# Autodesk Inventor assembly: Leg_joint_roll_yaw
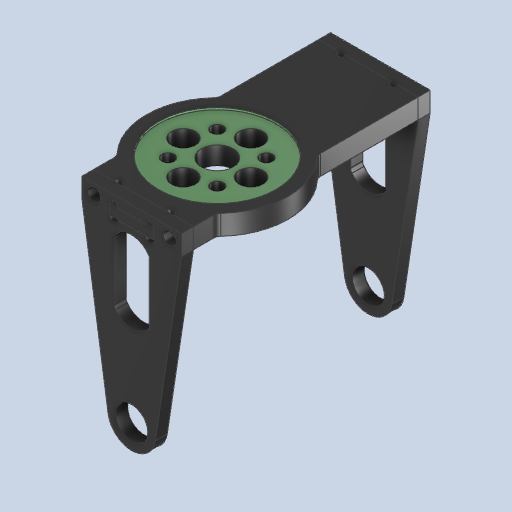
[picture p0: Inventor's stored thumbnail of the model, 512x512]
Saved by Autodesk Inventor 2022 (Build 260153000, 153)
## iProperties
Created: 2022-06-15
Part Number: Leg_joint_roll_yaw
Document SubType Name: Assembly
Designer: Masato Kubotera
Mass: 30.8099 g
Surface Area: 90.7098 cm^2
Volume: 11.0036 cm^3
Density: 2.8 g/cm^3
Author: Masato Kubotera
## Documents named in this file (6)
- C:\Users\MasatoKubotera\Documents\Inventor\SUSTAINA-OP\LowerBody\Leg_joint\Leg_joint_roll_yaw.iam
- C:\Users\MasatoKubotera\Documents\Inventor\SUSTAINA-OP\LowerBody\Leg_joint\Leg_joint_slider_frame.ipt
- C:\Users\MasatoKubotera\Documents\Inventor\SUSTAINA-OP\LowerBody\Leg_joint\Leg_joint_yaw_frame.ipt
- C:\Users\MasatoKubotera\Documents\Inventor\SUSTAINA-OP\ReadyMade\Screw\UC-0310.ipt
- C:\Users\MasatoKubotera\Documents\Inventor\SUSTAINA-OP\ReadyMade\Screw\UC-0306.ipt
- C:\Users\MasatoKubotera\Documents\Inventor\SUSTAINA-OP\LowerBody\Leg_joint\Leg_joint_roll_yaw_簡略化_1.ipt
## Components (11 placed, 4 different names)
1. Leg_joint_yaw_frame:1 — メイト:2, フラッシュ:2, フラッシュ:3, 挿入:1, 挿入:2, 挿入:3, 挿入:4, 挿入:5, 挿入:6, 挿入:7, 挿入:8
2. Leg_joint_slider_frame:1 — 挿入:1, 挿入:2, 挿入:9, 挿入:10
3. Leg_joint_slider_frame:2 — 挿入:3, 挿入:4, 挿入:11, 挿入:12
4. UC-0310:1 — 挿入:5
5. UC-0310:2 — 挿入:6
6. UC-0310:3 — 挿入:7
7. UC-0310:4 — 挿入:8
8. UC-0306:1 — 挿入:9
9. UC-0306:2 — 挿入:10
10. UC-0306:3 — 挿入:11
11. UC-0306:4 — 挿入:12
## Relationships (15: Insert 12, Flush 2, Mate 1)
- メイト:2 [Mate]: Leg_joint_yaw_frame:1
- フラッシュ:2 [Flush]: Leg_joint_yaw_frame:1
- フラッシュ:3 [Flush]: Leg_joint_yaw_frame:1
- 挿入:1 [Insert]: Leg_joint_yaw_frame:1 ↔ Leg_joint_slider_frame:1
- 挿入:2 [Insert]: Leg_joint_yaw_frame:1 ↔ Leg_joint_slider_frame:1
- 挿入:3 [Insert]: Leg_joint_yaw_frame:1 ↔ Leg_joint_slider_frame:2
- 挿入:4 [Insert]: Leg_joint_yaw_frame:1 ↔ Leg_joint_slider_frame:2
- 挿入:5 [Insert]: Leg_joint_yaw_frame:1 ↔ UC-0310:1
- 挿入:6 [Insert]: Leg_joint_yaw_frame:1 ↔ UC-0310:2
- 挿入:7 [Insert]: Leg_joint_yaw_frame:1 ↔ UC-0310:3
- 挿入:8 [Insert]: Leg_joint_yaw_frame:1 ↔ UC-0310:4
- 挿入:9 [Insert]: Leg_joint_slider_frame:1 ↔ UC-0306:1
- 挿入:10 [Insert]: Leg_joint_slider_frame:1 ↔ UC-0306:2
- 挿入:11 [Insert]: Leg_joint_slider_frame:2 ↔ UC-0306:3
- 挿入:12 [Insert]: Leg_joint_slider_frame:2 ↔ UC-0306:4
